(part 1 of 2)
# Autodesk Inventor assembly: NewChassis
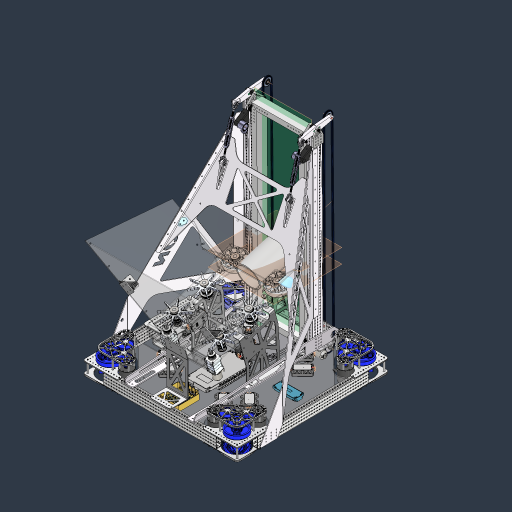
[picture p0: Inventor's stored thumbnail of the model, 512x512]
Saved by Autodesk Inventor 2024.3 (Build 283343000, 343)
## iProperties
ILogicPurgeVersion: 0.0.0.0
OnSaveVersion: 3.4.3.0
OnSaveAssembly: COREAutomationManager
Created: 2025-01-13
Part Number: NewChassis
Document SubType Name: Assembly
Designer: Marcus Tannini
Mfg Approved By: John.Thibert
Mass: 38555.3 g
Surface Area: 112070 cm^2
Volume: 16960.9 cm^3
Density: 2.27319 g/cm^3
ModelCat: Uncategorized
CN_MASS: 40.55
Author: Marcus Tannini
## Documents named in this file (68)
- C:\Users\Marcus Tannini\Documents\GitHub\2025-Poseidon-Mechanical\#Poseidon 2025.iam
- C:\Users\Marcus Tannini\Documents\GitHub\2025-Poseidon-Mechanical\ASSY,MK4i,Swerve_Module_INV.iam
- C:\Users\Marcus Tannini\Documents\GitHub\2025-Poseidon-Mechanical\MAXTube-2x1-Holes.ipt
- C:\Users\Marcus Tannini\Documents\GitHub\2025-Poseidon-Mechanical\BellyPanTop.ipt
- C:\Users\Marcus Tannini\Documents\GitHub\2025-Poseidon-Mechanical\BellyPanBot.ipt
- C:\Users\Marcus Tannini\Documents\GitHub\2025-Poseidon-Mechanical\BATTERY,12V.ipt
- C:\Users\Marcus Tannini\Documents\GitHub\2025-Poseidon-Mechanical\CONTROLS,MAIN_BREAKER.ipt
- C:\Users\Marcus Tannini\Documents\GitHub\2025-Poseidon-Mechanical\CONTROLS,MOTOR,NEO,550.ipt
- C:\Users\Marcus Tannini\Documents\GitHub\2025-Poseidon-Mechanical\CONTROLS,PDH.ipt
- C:\Users\Marcus Tannini\Documents\GitHub\2025-Poseidon-Mechanical\CONTROLS,PH.ipt
- C:\Users\Marcus Tannini\Documents\GitHub\2025-Poseidon-Mechanical\CONTROLS,ROBO_RIO.ipt
- C:\Users\Marcus Tannini\Documents\GitHub\2025-Poseidon-Mechanical\CONTROLS,SPARK_MAX.ipt
- C:\Users\Marcus Tannini\Documents\GitHub\2025-Poseidon-Mechanical\CONTROLS,VRM.ipt
- C:\Users\Marcus Tannini\Documents\GitHub\2025-Poseidon-Mechanical\COVER,SPARKMAX.ipt
- C:\Users\Marcus Tannini\Documents\GitHub\2025-Poseidon-Mechanical\ModifiedCase(IncludesPatterning).iam
- C:\Users\Marcus Tannini\Documents\GitHub\2025-Poseidon-Mechanical\PLATE,MOUNT,BATTERY,TOP.ipt
- C:\Users\Marcus Tannini\Documents\GitHub\2025-Poseidon-Mechanical\PLATE,MOUNT,BATTERY,BOT.ipt
- C:\Users\Marcus Tannini\Documents\GitHub\2025-Poseidon-Mechanical\MOUNT,STRAP,BATTERY.ipt
- C:\Users\Marcus Tannini\Documents\GitHub\2025-Poseidon-Mechanical\SPACER,SPROCKET,IDLER,ELEVATOR.ipt
- C:\Users\Marcus Tannini\Documents\GitHub\2025-Poseidon-Mechanical\22.ipt
- C:\Users\Marcus Tannini\Documents\GitHub\2025-Poseidon-Mechanical\PLATE,MOUNT,DRIVE,ELEVATOR.ipt
- C:\Users\Marcus Tannini\Documents\GitHub\2025-Poseidon-Mechanical\PLATE,BEARING,DRIVE,ELEVATOR.ipt
- C:\Users\Marcus Tannini\Documents\GitHub\2025-Poseidon-Mechanical\PURCHASED,HEX_BEARING.ipt
- C:\Users\Marcus Tannini\Documents\GitHub\2025-Poseidon-Mechanical\SHAFT,HEX,0.500in,DRIVE,ELEVATOR.ipt
- C:\Users\Marcus Tannini\Documents\GitHub\2025-Poseidon-Mechanical\PLATE,SIDE,BRACE,RIGHT,ELEVATOR.ipt
- C:\Users\Marcus Tannini\Documents\GitHub\2025-Poseidon-Mechanical\PLATE,SIDE,BRACE,LEFT,ELEVATOR.ipt
- C:\Users\Marcus Tannini\Documents\GitHub\2025-Poseidon-Mechanical\PLATE,TURNBUCKLE,TENSIONER,CHAIN.ipt
- C:\Users\Marcus Tannini\Documents\GitHub\2025-Poseidon-Mechanical\PLATE,BRACE,HORISONTAL,TOP,ELEVATOR.ipt
- C:\Users\Marcus Tannini\Documents\GitHub\2025-Poseidon-Mechanical\TURNBUCKLE,0.25IN_CLEVIS.iam
- C:\Users\Marcus Tannini\Documents\GitHub\2025-Poseidon-Mechanical\STAGE1,ELEVATOR.iam
- C:\Users\Marcus Tannini\Documents\GitHub\2025-Poseidon-Mechanical\ASSY,MAIN,ELEVATOR.iam
- C:\Users\Marcus Tannini\Documents\GitHub\2025-Poseidon-Mechanical\ANGLE,MOUNT,ELEVATOR.ipt
- C:\Users\Marcus Tannini\Documents\GitHub\2025-Poseidon-Mechanical\ANGLE,MOUNT,ELEVATOR,MIRR.ipt
- C:\Users\Marcus Tannini\Documents\GitHub\2025-Poseidon-Mechanical\FABRIC,BUMPERS.ipt
- C:\Users\Marcus Tannini\Documents\GitHub\2025-Poseidon-Mechanical\9293K119_Constant-Force Spring.ipt
- C:\Users\Marcus Tannini\Documents\GitHub\2025-Poseidon-Mechanical\MOUNT,SPRING,ELEVATOR.ipt
- C:\Users\Marcus Tannini\Documents\GitHub\2025-Poseidon-Mechanical\MOUNT,SPRING,ELEVATOR,MIRR.ipt
- C:\Users\Marcus Tannini\Documents\GitHub\2025-Poseidon-Mechanical\VersaPlanetary v2 Dual Stage 10_1 with RS 550 (1).iam
- C:\Users\Marcus Tannini\Documents\GitHub\2025-Poseidon-Mechanical\hopper_side_l.ipt
- C:\Users\Marcus Tannini\Documents\GitHub\2025-Poseidon-Mechanical\hopper_side_r.ipt
- C:\Users\Marcus Tannini\Documents\GitHub\2025-Poseidon-Mechanical\hopper_back.ipt
- C:\Users\Marcus Tannini\Documents\GitHub\2025-Poseidon-Mechanical\feeder_bottom_plate.ipt
- C:\Users\Marcus Tannini\Documents\GitHub\2025-Poseidon-Mechanical\hopper_side_bracket.ipt
- C:\Users\Marcus Tannini\Documents\GitHub\2025-Poseidon-Mechanical\feeder_guide_plate.ipt
- C:\Users\Marcus Tannini\Documents\GitHub\2025-Poseidon-Mechanical\am-5123 5IN 500IN Hex Bore Compliant Star.iam
- C:\Users\Marcus Tannini\Documents\GitHub\2025-Poseidon-Mechanical\feeder_guide_plate_MIR.ipt
- C:\Users\Marcus Tannini\Documents\GitHub\2025-Poseidon-Mechanical\feeder_front_support.ipt
- C:\Users\Marcus Tannini\Documents\GitHub\2025-Poseidon-Mechanical\Coral.ipt
- C:\Users\Marcus Tannini\Documents\GitHub\2025-Poseidon-Mechanical\coral_guide.ipt
- C:\Users\Marcus Tannini\Documents\GitHub\2025-Poseidon-Mechanical\coral_guide_MIR.ipt
- C:\Users\Marcus Tannini\Documents\GitHub\2025-Poseidon-Mechanical\hopper_back_support.ipt
- C:\Users\Marcus Tannini\Documents\GitHub\2025-Poseidon-Mechanical\feeder_side_support_r.ipt
- C:\Users\Marcus Tannini\Documents\GitHub\2025-Poseidon-Mechanical\feeder_side_support_l.ipt
- C:\Users\Marcus Tannini\Documents\GitHub\2025-Poseidon-Mechanical\feeder_middle_brace.ipt
- C:\Users\Marcus Tannini\Documents\GitHub\2025-Poseidon-Mechanical\2_1-2_hex_shaft.ipt
- C:\Users\Marcus Tannini\Documents\GitHub\2025-Poseidon-Mechanical\Bolt_Spacer.ipt
- C:\Users\Marcus Tannini\Documents\GitHub\2025-Poseidon-Mechanical\hopper_backboard.ipt
- C:\Users\Marcus Tannini\Documents\GitHub\2025-Poseidon-Mechanical\16t 9mm.ipt
- C:\Users\Marcus Tannini\Documents\GitHub\2025-Poseidon-Mechanical\19t 9mm.ipt
- C:\Users\Marcus Tannini\Documents\GitHub\2025-Poseidon-Mechanical\29t 9mm.ipt
- C:\Users\Marcus Tannini\Documents\GitHub\2025-Poseidon-Mechanical\coral_end_stop.ipt
- C:\Users\Marcus Tannini\Documents\GitHub\2025-Poseidon-Mechanical\coral_end_stop_MIR.ipt
- C:\Users\Marcus Tannini\Documents\GitHub\2025-Poseidon-Mechanical\Part Studio 1 - Support 1.ipt
- C:\Users\Marcus Tannini\Documents\GitHub\2025-Poseidon-Mechanical\Part Studio 1 - Support 2.ipt
- C:\Users\Marcus Tannini\Documents\GitHub\2025-Poseidon-Mechanical\am-3480 4IN 500Hex Bore Compliant Wheel REV2(1).iam
- C:\Users\Marcus Tannini\Documents\GitHub\2025-Poseidon-Mechanical\1-2in_spacer.ipt
- C:\Users\Marcus Tannini\Documents\GitHub\2025-Poseidon-Mechanical\hopper_fin.ipt
- C:\Users\Marcus Tannini\Documents\GitHub\2025-Poseidon-Mechanical\hopper_fin_MIR.ipt
## Components (143 placed, 70 different names)
1. FABRIC,BUMPERS.ipt:1 — Flush:323, Mate:335, Mate:336
2. am-3480 4IN 500Hex Bore Compliant Wheel REV2(1):1 [sub-assembly] — Mate:717, Mate:718, Mate:719, Mate:725
3. am-3480 4IN 500Hex Bore Compliant Wheel REV2(1):2 [sub-assembly] — Mate:720, Mate:721, Mate:722
4. 1-2in_spacer:1 — Mate:723, Mate:724, Mate:725
5. 1-2in_spacer:2 — Mate:726, Mate:727, Mate:728
6. 1-2in_spacer:3 — Mate:729, Mate:730, Mate:731
7. 1-2in_spacer:4 — Mate:738, Mate:739, Mate:740
8. 1-2in_spacer:5 — Mate:735, Mate:736, Mate:737
9. 1-2in_spacer:6 — Mate:732, Mate:733, Mate:734
10. hopper_fin:1 — Mate:749, Mate:750, Mate:754
11. hopper_fin_MIR:1 — Mate:751, Mate:752, Mate:753
12. BellyPanBot.ipt:1 — Mate:66, Mate:353, Mate:354
13. BellyPanTop.ipt:1 — Mate:62, Mate:63, Mate:65, Mate:70, Mate:71, Mate:82, Mate:84, Insert:7, Insert:8, Insert:9, Insert:10, Insert:11, Insert:12, Insert:13, Insert:14, Insert:15, Insert:16, Insert:17, Insert:18, Insert:19, Insert:20, Insert:21, Insert:22, Mate:111, Mate:113, Mate:114, Mate:116, Mate:117, Mate:118, Mate:119, Mate:121, Mate:122, Mate:123, Mate:124, Mate:125, Mate:126, Mate:127, Mate:130, Insert:23, Insert:24, Mate:223, Mate:308, Mate:320, Mate:349, Mate:350, Angle:11, Mate:541, Mate:542, Mate:544, Mate:548, Flush:336, Mate:549
14. MAXTube-2x1-Holes.ipt:1 — Mate:1, Mate:2, Mate:3, Mate:4, Mate:5, Mate:15, Mate:115, Mate:272
15. MAXTube-2x1-Holes.ipt:2 — Mate:6, Mate:7, Mate:8, Mate:9, Mate:10, Mate:11, Mate:62, Flush:17, Mate:309, Mate:310, Mate:542, Mate:543
16. MAXTube-2x1-Holes.ipt:3 — Mate:19, Mate:20, Mate:21, Mate:66, Mate:114, Mate:312, Mate:313, Mate:336
17. MAXTube-2x1-Holes.ipt:4 — Mate:12, Mate:13, Mate:14, Mate:16, Mate:17, Mate:18, Mate:29, Mate:63, Mate:271, Mate:353, Mate:354
18. MOUNT,STRAP,BATTERY.ipt:1 — Mate:357, Mate:358, Mate:359
19. PLATE,MOUNT,BATTERY,BOT.ipt:1 — Mate:320, Mate:321, Mate:351, Mate:352
20. PLATE,MOUNT,BATTERY,TOP.ipt:1 — Mate:127, Mate:349, Mate:350, Mate:351, Mate:352, Mate:356, Mate:357, Mate:358, Mate:359
21. BATTERY,12V.ipt:1 — Mate:321, Mate:356
22. CONTROLS,MAIN_BREAKER.ipt:1 — Mate:82, Mate:111, Mate:116
23. CONTROLS,PDH.ipt:1 — Mate:113, Mate:117, Mate:118, Mate:119
24. CONTROLS,PH.ipt:1 — Insert:23, Insert:24
25. CONTROLS,ROBO_RIO.ipt:1 — Mate:124, Mate:125, Mate:126
26. CONTROLS,SPARK_MAX.ipt:1 — Mate:84, Mate:85, Mate:86, Mate:87
27. CONTROLS,VRM.ipt:1 — Mate:121, Mate:122, Mate:123
28. ModifiedCase(IncludesPatterning).iam:1 [sub-assembly] — Mate:130
29. ASSY,MK4i,Swerve_Module_INV.iam:1 [sub-assembly] — Mate:1, Mate:2, Mate:15
30. ASSY,MK4i,Swerve_Module_INV.iam:2 [sub-assembly] — Mate:3, Mate:4, Mate:5, Mate:6, Mate:7, Mate:8
31. ASSY,MK4i,Swerve_Module_INV.iam:3 [sub-assembly] — Mate:9, Mate:10, Mate:11, Mate:12, Mate:13, Mate:14
32. ASSY,MK4i,Swerve_Module_INV.iam:4 [sub-assembly] — Mate:16, Mate:17, Mate:18, Mate:19, Mate:20, Mate:21, Mate:67
33. CONTROLS,SPARK_MAX.ipt:2
34. CONTROLS,SPARK_MAX.ipt:3
35. CONTROLS,SPARK_MAX.ipt:4
36. CONTROLS,SPARK_MAX.ipt:5
37. CONTROLS,SPARK_MAX.ipt:6
38. CONTROLS,SPARK_MAX.ipt:7
39. CONTROLS,SPARK_MAX.ipt:8
40. COVER,SPARKMAX.ipt:1 — Mate:85, Mate:86, Mate:87, Insert:7, Insert:8
41. COVER,SPARKMAX.ipt:2 — Insert:9, Insert:10
42. COVER,SPARKMAX.ipt:3 — Insert:11, Insert:12
43. COVER,SPARKMAX.ipt:4 — Insert:13, Insert:14
44. COVER,SPARKMAX.ipt:5 — Insert:17, Insert:18
45. COVER,SPARKMAX.ipt:6 — Insert:15, Insert:16
46. COVER,SPARKMAX.ipt:7 — Insert:21, Insert:22
47. COVER,SPARKMAX.ipt:8 — Insert:19, Insert:20
48. 9293K119_Constant-Force Spring:1 — Mate:364, Mate:365
49. 9293K119_Constant-Force Spring:2 — Mate:370, Mate:371
50. MOUNT,SPRING,ELEVATOR:1 — Mate:363, Mate:362, Mate:364, Mate:365, Mate:366
51. MOUNT,SPRING,ELEVATOR,MIRR:1 — Mate:367, Mate:368, Mate:369, Mate:370, Mate:371
52. CONTROLS,MOTOR,NEO,550:3
53. VersaPlanetary v2 Dual Stage 10_1 with RS 550 (1):1 [sub-assembly] — Mate:472, Mate:473, Mate:474
54. CONTROLS,MOTOR,NEO,550:4
55. VersaPlanetary v2 Dual Stage 10_1 with RS 550 (1):2 [sub-assembly] — Mate:469, Mate:470, Mate:471
56. ASSY,MAIN,ELEVATOR.iam:1 [sub-assembly] — Mate:161, Mate:162, Flush:19, Mate:297, STAGE1 UPPER LIMIT, STAGE1 MAX, Mate:311, Mate:314, Mate:315, Mate:363, Mate:362, Mate:366, Mate:367, Mate:368, Mate:369
57. STAGE1,ELEVATOR.iam:1 [sub-assembly] — Flush:19, Mate:297, STAGE1 LOWER LIMIT, STAGE1 UPPER LIMIT, STAGE1 MIN, STAGE1 MAX
58. 22.ipt:1 — Mate:227, Angle:6
59. 22.ipt:2 — Mate:233, Angle:4, Flush:14
60. ANGLE,MOUNT,ELEVATOR.ipt:1 — Mate:65, Mate:70, Mate:71, Mate:161, Mate:162, Mate:224, STAGE1 LOWER LIMIT, STAGE1 MIN, Flush:337, Mate:556
61. ANGLE,MOUNT,ELEVATOR,MIRR.ipt:1 — Mate:308, Mate:309, Mate:310, Mate:311, Mate:312, Mate:313, Mate:314, Mate:315, Flush:329, Angle:12, Mate:550, Mate:551, Mate:552
62. PLATE,BEARING,DRIVE,ELEVATOR.ipt:1 — Mate:226, Mate:227, Mate:228, Mate:229, Insert:50
63. PLATE,BEARING,DRIVE,ELEVATOR.ipt:2 — Mate:230, Mate:231, Mate:232, Insert:49, Mate:233, Mate:234
64. PLATE,BRACE,HORISONTAL,TOP,ELEVATOR.ipt:1 — Mate:285, Mate:286, Mate:289, Mate:290, Mate:291, Mate:295, Mate:296, Mate:714, Mate:746, Mate:747, Mate:748
65. PLATE,MOUNT,DRIVE,ELEVATOR.ipt:1 — Mate:223, Mate:224, Mate:226, Mate:228, Mate:229, Mate:230, Mate:231, Mate:232, Flush:329, Mate:469, Mate:470, Mate:471, Mate:472, Mate:473, Mate:474
66. PLATE,SIDE,BRACE,LEFT,ELEVATOR.ipt:1 — Mate:271, Mate:289, Mate:290, Mate:291, Mate:335
67. PLATE,SIDE,BRACE,RIGHT,ELEVATOR.ipt:1 — Mate:272
68. PLATE,TURNBUCKLE,TENSIONER,CHAIN.ipt:1 — Mate:285, Mate:296
69. PLATE,TURNBUCKLE,TENSIONER,CHAIN.ipt:2 — Mate:286, Mate:295
70. PURCHASED,HEX_BEARING.ipt:1 — Insert:49, Angle:5
71. PURCHASED,HEX_BEARING.ipt:2 — Insert:50, Angle:7
72. SHAFT,HEX,0.500in,DRIVE,ELEVATOR.ipt:1 — Mate:234, Angle:4, Angle:5, Angle:6, Angle:7, Flush:14
73. SPACER,SPROCKET,IDLER,ELEVATOR.ipt:1
74. SPACER,SPROCKET,IDLER,ELEVATOR.ipt:2
75. TURNBUCKLE,0.25IN_CLEVIS.iam:1 [sub-assembly]
76. TURNBUCKLE,0.25IN_CLEVIS.iam:2 [sub-assembly]
77. Part Studio 1 - Support 2:1 — Mate:743, Mate:744, Mate:745
78. Part Studio 1 - Support 1:1 — Mate:713, Mate:714
79. coral_end_stop_MIR:1 — Flush:364, Mate:715, Flush:365
80. coral_end_stop:1 — Mate:704, Flush:362, Flush:364, Mate:715, Flush:365, Mate:716
81. hopper_side_l:1 — Mate:496, Mate:497, Mate:498, Mate:743, Mate:744, Mate:745
82. hopper_side_r:1 — Mate:502, Mate:503, Mate:504, Mate:713
83. feeder_bottom_plate:1 — Angle:11, Mate:490, Mate:491, Mate:492, Mate:507, Mate:512, Mate:519, Mate:534, Angle:12, Flush:333, Mate:537, Flush:334, Mate:539, Flush:335, Mate:545, Mate:546, Mate:547, Mate:577, Mate:578, Mate:605, Mate:608, Mate:609, Mate:610, Mate:611, Mate:630, Mate:631, Mate:632, Mate:633, Mate:634, Mate:646, Mate:647, Mate:648, Mate:649, Mate:656, Mate:657, Mate:658, Mate:659, Mate:698, Mate:700, Mate:741, Mate:742
84. hopper_back:1 — Mate:490, Mate:491, Mate:492, Mate:493, Mate:494, Mate:495, Mate:499, Mate:500, Mate:501, Mate:749, Mate:750, Mate:751, Mate:752, Mate:753, Mate:754
85. hopper_side_bracket:1 — Mate:493, Mate:494, Mate:495, Mate:496, Mate:497, Mate:498
86. hopper_side_bracket:2 — Mate:499, Mate:500, Mate:501, Mate:502, Mate:503, Mate:504
87. feeder_guide_plate:1 — Mate:507, Mate:577, Mate:644, Mate:645, Mate:650, Mate:651, Mate:652, Mate:653, Mate:699, Mate:742
88. am-5123 5IN 500IN Hex Bore Compliant Star:2 [sub-assembly] — Flush:353, Mate:654, Mate:655, Flush:354, Mate:731
89. feeder_guide_plate_MIR:1 — Mate:512, Mate:520, Mate:578, Mate:660, Mate:661, Mate:662, Mate:663, Mate:664, Mate:665, Mate:701, Mate:741
90. feeder_front_support:1 — Mate:541, Mate:543, Mate:544, Mate:704, Flush:362, Mate:716
91. Coral:1 — Mate:519, Mate:520, Mate:630
92. CONTROLS,MOTOR,NEO,550:5
93. VersaPlanetary v2 Dual Stage 10_1 with RS 550 (1):3 [sub-assembly] — Mate:534, Mate:631, Mate:632, Mate:668, Mate:670
94. coral_guide:1 — Flush:333, Mate:537, Mate:540, Flush:335
95. coral_guide_MIR:1 — Flush:334, Mate:539, Mate:540
96. hopper_back_support:1 — Mate:545, Mate:546, Mate:547, Mate:548, Flush:336, Mate:549
97. feeder_side_support_r:1 — Flush:337, Mate:553, Mate:554, Mate:555, Mate:556, Mate:624, Mate:625, Mate:626
98. feeder_side_support_l:1 — Mate:550, Mate:551, Mate:552, Mate:627, Mate:628, Mate:629
99. feeder_middle_brace:1 — Mate:553, Mate:554, Mate:555
100. 2_1-2_hex_shaft:1 — Mate:557, Mate:558, Flush:340, Mate:561, Mate:562, Rotation:4, Rotation:5, Mate:685, Mate:686, Mate:688, Mate:689, Mate:726, Mate:727
101. PURCHASED,HEX_BEARING:3 — Mate:557, Mate:558, Flush:340, Mate:573, Mate:652, Mate:653
102. 2_1-2_hex_shaft:2 — Rotation:5, Mate:690, Mate:691, Mate:717, Mate:718, Mate:723, Mate:724
103. PURCHASED,HEX_BEARING:4 — Mate:650, Mate:651, Mate:719
104. am-5123 5IN 500IN Hex Bore Compliant Star:3 [sub-assembly] — Mate:561, Mate:562, Mate:573, Flush:353
105. 2_1-2_hex_shaft:3 — Rotation:1, Rotation:2, Mate:680, Mate:681, Mate:693, Mate:694, Mate:735, Mate:736
106. PURCHASED,HEX_BEARING:5 — Mate:660, Mate:661
107. am-5123 5IN 500IN Hex Bore Compliant Star:5 [sub-assembly]
108. 2_1-2_hex_shaft:4 — Rotation:2, Mate:695, Mate:696, Mate:720, Mate:721, Mate:738, Mate:739
109. PURCHASED,HEX_BEARING:6 — Mate:662, Mate:663, Mate:722
110. am-5123 5IN 500IN Hex Bore Compliant Star:7 [sub-assembly] — Mate:666, Mate:667, Flush:354
111. CONTROLS,MOTOR,NEO,550:6
112. VersaPlanetary v2 Dual Stage 10_1 with RS 550 (1):4 [sub-assembly] — Mate:605, Mate:633, Mate:634, Mate:673, Mate:674
113. PURCHASED,HEX_BEARING:7 — Mate:648, Mate:649
114. PURCHASED,HEX_BEARING:8 — Mate:646, Mate:647
115. PURCHASED,HEX_BEARING:9 — Mate:658, Mate:659
116. PURCHASED,HEX_BEARING:10 — Mate:656, Mate:657
117. Bolt_Spacer:1 — Mate:608, Mate:609
118. Bolt_Spacer:2 — Mate:610, Mate:611
119. hopper_backboard:1 — Mate:746, Mate:747, Mate:748
120. CONTROLS,SPARK_MAX:9 — Mate:626
121. COVER,SPARKMAX:9 — Mate:624, Mate:625
122. CONTROLS,SPARK_MAX:10 — Mate:629
123. COVER,SPARKMAX:10 — Mate:627, Mate:628
124. PURCHASED,HEX_BEARING:11 — Mate:636, Mate:637, Flush:349, Mate:664, Mate:665
125. 2_1-2_hex_shaft:5 — Flush:351, Mate:640, Mate:641, Flush:352, Mate:642, Mate:643, Mate:654, Mate:655, Rotation:3, Rotation:4, Mate:671, Mate:672, Mate:682, Mate:684, Mate:729, Mate:730
126. 2_1-2_hex_shaft:6 — Mate:636, Mate:637, Flush:349, Flush:350, Mate:638, Mate:639, Mate:666, Mate:667, Rotation:1, Rotation:3, Mate:675, Mate:676, Mate:678, Mate:679, Mate:732, Mate:733
127. PURCHASED,HEX_BEARING:12 — Flush:351, Mate:640, Mate:641, Mate:644, Mate:645
128. PURCHASED,HEX_BEARING:13 — Flush:352, Mate:642, Mate:643
129. PURCHASED,HEX_BEARING:14 — Flush:350, Mate:638, Mate:639, Mate:697
130. 16t 9mm:1 — Mate:671, Mate:672, Flush:355, Mate:683
131. 16t 9mm:2 — Mate:668, Mate:670, Flush:355, Flush:356
132. 16t 9mm:3 — Mate:673, Mate:674, Flush:356, Flush:357
133. 16t 9mm:4 — Mate:675, Mate:676, Flush:357, Mate:677, Mate:697
134. 19t 9mm:1 — Mate:682, Mate:683, Mate:684, Flush:359
135. 19t 9mm:2 — Mate:680, Flush:358, Mate:681, Mate:692, Mate:737
136. 19t 9mm:3 — Mate:678, Mate:677, Mate:679, Flush:358, Mate:734
137. 19t 9mm:4 — Mate:685, Flush:359, Mate:686, Mate:687, Mate:728
138. 29t 9mm:1 — Flush:360, Mate:690, Mate:691
139. 29t 9mm:2 — Mate:687, Mate:688, Mate:689, Flush:360
140. 29t 9mm:3 — Mate:692, Mate:693, Mate:694, Flush:361
141. 29t 9mm:4 — Flush:361, Mate:695, Mate:696, Mate:740
142. Bolt_Spacer:3 — Mate:698, Mate:699
143. Bolt_Spacer:4 — Mate:700, Mate:701
## Relationships (411: Mate 342, Flush 34, Insert 24, Angle 6, RelateRotation 5)
- Mate:1: MAXTube-2x1-Holes.ipt:1 ↔ ASSY,MK4i,Swerve_Module_INV.iam:1
- Mate:2: MAXTube-2x1-Holes.ipt:1 ↔ ASSY,MK4i,Swerve_Module_INV.iam:1
- Mate:3: MAXTube-2x1-Holes.ipt:1 ↔ ASSY,MK4i,Swerve_Module_INV.iam:2
- Mate:4: MAXTube-2x1-Holes.ipt:1 ↔ ASSY,MK4i,Swerve_Module_INV.iam:2
- Mate:5: MAXTube-2x1-Holes.ipt:1 ↔ ASSY,MK4i,Swerve_Module_INV.iam:2
- Mate:6: MAXTube-2x1-Holes.ipt:2 ↔ ASSY,MK4i,Swerve_Module_INV.iam:2
- Mate:7: MAXTube-2x1-Holes.ipt:2 ↔ ASSY,MK4i,Swerve_Module_INV.iam:2
- Mate:8: MAXTube-2x1-Holes.ipt:2 ↔ ASSY,MK4i,Swerve_Module_INV.iam:2
- Mate:9: MAXTube-2x1-Holes.ipt:2 ↔ ASSY,MK4i,Swerve_Module_INV.iam:3
- Mate:10: MAXTube-2x1-Holes.ipt:2 ↔ ASSY,MK4i,Swerve_Module_INV.iam:3
- Mate:11: MAXTube-2x1-Holes.ipt:2 ↔ ASSY,MK4i,Swerve_Module_INV.iam:3
- Mate:12: MAXTube-2x1-Holes.ipt:4 ↔ ASSY,MK4i,Swerve_Module_INV.iam:3
- Mate:13: MAXTube-2x1-Holes.ipt:4 ↔ ASSY,MK4i,Swerve_Module_INV.iam:3
- Mate:14: MAXTube-2x1-Holes.ipt:4 ↔ ASSY,MK4i,Swerve_Module_INV.iam:3
- Mate:15: MAXTube-2x1-Holes.ipt:1 ↔ ASSY,MK4i,Swerve_Module_INV.iam:1
- Mate:16: MAXTube-2x1-Holes.ipt:4 ↔ ASSY,MK4i,Swerve_Module_INV.iam:4
- Mate:17: MAXTube-2x1-Holes.ipt:4 ↔ ASSY,MK4i,Swerve_Module_INV.iam:4
- Mate:18: MAXTube-2x1-Holes.ipt:4 ↔ ASSY,MK4i,Swerve_Module_INV.iam:4
- Mate:19: MAXTube-2x1-Holes.ipt:3 ↔ ASSY,MK4i,Swerve_Module_INV.iam:4
- Mate:20: MAXTube-2x1-Holes.ipt:3 ↔ ASSY,MK4i,Swerve_Module_INV.iam:4
- Mate:21: MAXTube-2x1-Holes.ipt:3 ↔ ASSY,MK4i,Swerve_Module_INV.iam:4
- Mate:29 (-6.35 mm): MAXTube-2x1-Holes.ipt:4
- Mate:62: BellyPanTop.ipt:1 ↔ MAXTube-2x1-Holes.ipt:2
- Mate:63: BellyPanTop.ipt:1 ↔ MAXTube-2x1-Holes.ipt:4
- Mate:65: BellyPanTop.ipt:1 ↔ ANGLE,MOUNT,ELEVATOR.ipt:1
- Mate:66: BellyPanBot.ipt:1 ↔ MAXTube-2x1-Holes.ipt:3
- Mate:67 (35.56 mm): ASSY,MK4i,Swerve_Module_INV.iam:4
- Mate:70: BellyPanTop.ipt:1 ↔ ANGLE,MOUNT,ELEVATOR.ipt:1
- Mate:71: BellyPanTop.ipt:1 ↔ ANGLE,MOUNT,ELEVATOR.ipt:1
- Mate:321: PLATE,MOUNT,BATTERY,BOT.ipt:1 ↔ BATTERY,12V.ipt:1
- Mate:82: BellyPanTop.ipt:1 ↔ CONTROLS,MAIN_BREAKER.ipt:1
- Mate:84: BellyPanTop.ipt:1 ↔ CONTROLS,SPARK_MAX.ipt:1
- Mate:85: CONTROLS,SPARK_MAX.ipt:1 ↔ COVER,SPARKMAX.ipt:1
- Mate:86: CONTROLS,SPARK_MAX.ipt:1 ↔ COVER,SPARKMAX.ipt:1
- Mate:87: CONTROLS,SPARK_MAX.ipt:1 ↔ COVER,SPARKMAX.ipt:1
- Insert:7: BellyPanTop.ipt:1 ↔ COVER,SPARKMAX.ipt:1
- Insert:8: BellyPanTop.ipt:1 ↔ COVER,SPARKMAX.ipt:1
- [Mate]: CONTROLS,SPARK_MAX.ipt:2 ↔ COVER,SPARKMAX.ipt:2
- [Mate]: CONTROLS,SPARK_MAX.ipt:2 ↔ COVER,SPARKMAX.ipt:2
- [Mate]: CONTROLS,SPARK_MAX.ipt:2 ↔ COVER,SPARKMAX.ipt:2
- [Mate]: CONTROLS,SPARK_MAX.ipt:3 ↔ COVER,SPARKMAX.ipt:3
- [Mate]: CONTROLS,SPARK_MAX.ipt:3 ↔ COVER,SPARKMAX.ipt:3
- [Mate]: CONTROLS,SPARK_MAX.ipt:3 ↔ COVER,SPARKMAX.ipt:3
- [Mate]: CONTROLS,SPARK_MAX.ipt:4 ↔ COVER,SPARKMAX.ipt:4
- [Mate]: CONTROLS,SPARK_MAX.ipt:4 ↔ COVER,SPARKMAX.ipt:4
- [Mate]: CONTROLS,SPARK_MAX.ipt:4 ↔ COVER,SPARKMAX.ipt:4
- [Mate]: CONTROLS,SPARK_MAX.ipt:5 ↔ COVER,SPARKMAX.ipt:5
- [Mate]: CONTROLS,SPARK_MAX.ipt:5 ↔ COVER,SPARKMAX.ipt:5
- [Mate]: CONTROLS,SPARK_MAX.ipt:5 ↔ COVER,SPARKMAX.ipt:5
- [Mate]: CONTROLS,SPARK_MAX.ipt:6 ↔ COVER,SPARKMAX.ipt:6
- [Mate]: CONTROLS,SPARK_MAX.ipt:6 ↔ COVER,SPARKMAX.ipt:6
- [Mate]: CONTROLS,SPARK_MAX.ipt:6 ↔ COVER,SPARKMAX.ipt:6
- [Mate]: CONTROLS,SPARK_MAX.ipt:7 ↔ COVER,SPARKMAX.ipt:7
- [Mate]: CONTROLS,SPARK_MAX.ipt:7 ↔ COVER,SPARKMAX.ipt:7
- [Mate]: CONTROLS,SPARK_MAX.ipt:7 ↔ COVER,SPARKMAX.ipt:7
- [Mate]: CONTROLS,SPARK_MAX.ipt:8 ↔ COVER,SPARKMAX.ipt:8
- [Mate]: CONTROLS,SPARK_MAX.ipt:8 ↔ COVER,SPARKMAX.ipt:8
- [Mate]: CONTROLS,SPARK_MAX.ipt:8 ↔ COVER,SPARKMAX.ipt:8
- Insert:9: BellyPanTop.ipt:1 ↔ COVER,SPARKMAX.ipt:2
- Insert:10: BellyPanTop.ipt:1 ↔ COVER,SPARKMAX.ipt:2
- Insert:11: BellyPanTop.ipt:1 ↔ COVER,SPARKMAX.ipt:3
- Insert:12: BellyPanTop.ipt:1 ↔ COVER,SPARKMAX.ipt:3
- Insert:13: BellyPanTop.ipt:1 ↔ COVER,SPARKMAX.ipt:4
- Insert:14: BellyPanTop.ipt:1 ↔ COVER,SPARKMAX.ipt:4
- Insert:15: BellyPanTop.ipt:1 ↔ COVER,SPARKMAX.ipt:6
- Insert:16: BellyPanTop.ipt:1 ↔ COVER,SPARKMAX.ipt:6
- Insert:17: BellyPanTop.ipt:1 ↔ COVER,SPARKMAX.ipt:5
- Insert:18: BellyPanTop.ipt:1 ↔ COVER,SPARKMAX.ipt:5
- Insert:19: BellyPanTop.ipt:1 ↔ COVER,SPARKMAX.ipt:8
- Insert:20: BellyPanTop.ipt:1 ↔ COVER,SPARKMAX.ipt:8
- Insert:21: BellyPanTop.ipt:1 ↔ COVER,SPARKMAX.ipt:7
- Insert:22: BellyPanTop.ipt:1 ↔ COVER,SPARKMAX.ipt:7
- Mate:111: BellyPanTop.ipt:1 ↔ CONTROLS,MAIN_BREAKER.ipt:1
- Mate:113: BellyPanTop.ipt:1 ↔ CONTROLS,PDH.ipt:1
- Mate:114: BellyPanTop.ipt:1 ↔ MAXTube-2x1-Holes.ipt:3
- Mate:115 (-374.65 mm): MAXTube-2x1-Holes.ipt:1
- Mate:116 (0.254 mm): BellyPanTop.ipt:1 ↔ CONTROLS,MAIN_BREAKER.ipt:1
- Mate:117: BellyPanTop.ipt:1 ↔ CONTROLS,PDH.ipt:1
- Mate:118: BellyPanTop.ipt:1 ↔ CONTROLS,PDH.ipt:1
- Mate:119: BellyPanTop.ipt:1 ↔ CONTROLS,PDH.ipt:1
- Mate:121: BellyPanTop.ipt:1 ↔ CONTROLS,VRM.ipt:1
- Mate:122: BellyPanTop.ipt:1 ↔ CONTROLS,VRM.ipt:1
- Mate:123: BellyPanTop.ipt:1 ↔ CONTROLS,VRM.ipt:1
- Mate:124: BellyPanTop.ipt:1 ↔ CONTROLS,ROBO_RIO.ipt:1
- Mate:125: BellyPanTop.ipt:1 ↔ CONTROLS,ROBO_RIO.ipt:1
- Mate:126: BellyPanTop.ipt:1 ↔ CONTROLS,ROBO_RIO.ipt:1
- Mate:127: BellyPanTop.ipt:1 ↔ PLATE,MOUNT,BATTERY,TOP.ipt:1
- Mate:130: BellyPanTop.ipt:1 ↔ ModifiedCase(IncludesPatterning).iam:1
- Insert:23: BellyPanTop.ipt:1 ↔ CONTROLS,PH.ipt:1
- Insert:24: BellyPanTop.ipt:1 ↔ CONTROLS,PH.ipt:1
- Mate:161: ASSY,MAIN,ELEVATOR.iam:1 ↔ ANGLE,MOUNT,ELEVATOR.ipt:1
- Mate:162: ASSY,MAIN,ELEVATOR.iam:1 ↔ ANGLE,MOUNT,ELEVATOR.ipt:1
- [Mate]: ASSY,MAIN,ELEVATOR.iam:1 ↔ ANGLE,MOUNT,ELEVATOR.ipt:1
- [Insert]: ASSY,MAIN,ELEVATOR.iam:1 ↔ SPACER,SPROCKET,IDLER,ELEVATOR.ipt:1
- [Insert]: ASSY,MAIN,ELEVATOR.iam:1 ↔ SPACER,SPROCKET,IDLER,ELEVATOR.ipt:1
- [Flush]: ASSY,MAIN,ELEVATOR.iam:1 ↔ 22.ipt:1
- [Insert]: ASSY,MAIN,ELEVATOR.iam:1 ↔ SPACER,SPROCKET,IDLER,ELEVATOR.ipt:2
- [Insert]: ASSY,MAIN,ELEVATOR.iam:1 ↔ SPACER,SPROCKET,IDLER,ELEVATOR.ipt:2
- Mate:223: BellyPanTop.ipt:1 ↔ PLATE,MOUNT,DRIVE,ELEVATOR.ipt:1
- Mate:224: ANGLE,MOUNT,ELEVATOR.ipt:1 ↔ PLATE,MOUNT,DRIVE,ELEVATOR.ipt:1
- Mate:226: PLATE,BEARING,DRIVE,ELEVATOR.ipt:1 ↔ PLATE,MOUNT,DRIVE,ELEVATOR.ipt:1
- Mate:227: 22.ipt:1 ↔ PLATE,BEARING,DRIVE,ELEVATOR.ipt:1
- Mate:228: PLATE,BEARING,DRIVE,ELEVATOR.ipt:1 ↔ PLATE,MOUNT,DRIVE,ELEVATOR.ipt:1
- Mate:229: PLATE,BEARING,DRIVE,ELEVATOR.ipt:1 ↔ PLATE,MOUNT,DRIVE,ELEVATOR.ipt:1
- Mate:230: PLATE,BEARING,DRIVE,ELEVATOR.ipt:2 ↔ PLATE,MOUNT,DRIVE,ELEVATOR.ipt:1
- Mate:231: PLATE,BEARING,DRIVE,ELEVATOR.ipt:2 ↔ PLATE,MOUNT,DRIVE,ELEVATOR.ipt:1
- Mate:232: PLATE,BEARING,DRIVE,ELEVATOR.ipt:2 ↔ PLATE,MOUNT,DRIVE,ELEVATOR.ipt:1
- Insert:49: PLATE,BEARING,DRIVE,ELEVATOR.ipt:2 ↔ PURCHASED,HEX_BEARING.ipt:1
- Insert:50: PLATE,BEARING,DRIVE,ELEVATOR.ipt:1 ↔ PURCHASED,HEX_BEARING.ipt:2
- Mate:233: 22.ipt:2 ↔ PLATE,BEARING,DRIVE,ELEVATOR.ipt:2
- Mate:234: PLATE,BEARING,DRIVE,ELEVATOR.ipt:2 ↔ SHAFT,HEX,0.500in,DRIVE,ELEVATOR.ipt:1
- Angle:4 (0 deg): 22.ipt:2 ↔ SHAFT,HEX,0.500in,DRIVE,ELEVATOR.ipt:1
- Angle:5 (0 deg): PURCHASED,HEX_BEARING.ipt:1 ↔ SHAFT,HEX,0.500in,DRIVE,ELEVATOR.ipt:1
- Angle:6 (0 deg): 22.ipt:1 ↔ SHAFT,HEX,0.500in,DRIVE,ELEVATOR.ipt:1
- Angle:7 (0 deg): PURCHASED,HEX_BEARING.ipt:2 ↔ SHAFT,HEX,0.500in,DRIVE,ELEVATOR.ipt:1
- [Flush]: ASSY,MAIN,ELEVATOR.iam:1 ↔ 22.ipt:2
- [Mate]: ASSY,MAIN,ELEVATOR.iam:1 ↔ PLATE,SIDE,BRACE,LEFT,ELEVATOR.ipt:1
- [Mate]: ASSY,MAIN,ELEVATOR.iam:1 ↔ PLATE,SIDE,BRACE,LEFT,ELEVATOR.ipt:1
- [Mate]: ASSY,MAIN,ELEVATOR.iam:1 ↔ 22.ipt:1
- Flush:14 (-15.875 mm): 22.ipt:2 ↔ SHAFT,HEX,0.500in,DRIVE,ELEVATOR.ipt:1
- Flush:17 (457.2 mm): MAXTube-2x1-Holes.ipt:2
- [Mate]: ASSY,MAIN,ELEVATOR.iam:1 ↔ PLATE,SIDE,BRACE,LEFT,ELEVATOR.ipt:1
- [Mate]: ASSY,MAIN,ELEVATOR.iam:1 ↔ PLATE,SIDE,BRACE,RIGHT,ELEVATOR.ipt:1
- [Mate]: ASSY,MAIN,ELEVATOR.iam:1 ↔ PLATE,SIDE,BRACE,RIGHT,ELEVATOR.ipt:1
- [Mate]: ASSY,MAIN,ELEVATOR.iam:1 ↔ PLATE,SIDE,BRACE,RIGHT,ELEVATOR.ipt:1
- Mate:271: MAXTube-2x1-Holes.ipt:4 ↔ PLATE,SIDE,BRACE,LEFT,ELEVATOR.ipt:1
- Mate:272: MAXTube-2x1-Holes.ipt:1 ↔ PLATE,SIDE,BRACE,RIGHT,ELEVATOR.ipt:1
- [Mate]: ASSY,MAIN,ELEVATOR.iam:1 ↔ TURNBUCKLE,0.25IN_CLEVIS.iam:1
- [Mate]: ASSY,MAIN,ELEVATOR.iam:1 ↔ TURNBUCKLE,0.25IN_CLEVIS.iam:1
- [Mate]: ASSY,MAIN,ELEVATOR.iam:1 ↔ TURNBUCKLE,0.25IN_CLEVIS.iam:2
- [Mate]: ASSY,MAIN,ELEVATOR.iam:1 ↔ TURNBUCKLE,0.25IN_CLEVIS.iam:2
- Mate:285: PLATE,BRACE,HORISONTAL,TOP,ELEVATOR.ipt:1 ↔ PLATE,TURNBUCKLE,TENSIONER,CHAIN.ipt:1
- Mate:286: PLATE,BRACE,HORISONTAL,TOP,ELEVATOR.ipt:1 ↔ PLATE,TURNBUCKLE,TENSIONER,CHAIN.ipt:2
- Mate:289: PLATE,BRACE,HORISONTAL,TOP,ELEVATOR.ipt:1 ↔ PLATE,SIDE,BRACE,LEFT,ELEVATOR.ipt:1
- Mate:290: PLATE,BRACE,HORISONTAL,TOP,ELEVATOR.ipt:1 ↔ PLATE,SIDE,BRACE,LEFT,ELEVATOR.ipt:1
- Mate:291: PLATE,BRACE,HORISONTAL,TOP,ELEVATOR.ipt:1 ↔ PLATE,SIDE,BRACE,LEFT,ELEVATOR.ipt:1
- [Mate]: ASSY,MAIN,ELEVATOR.iam:1 ↔ 22.ipt:2
- Mate:295: PLATE,BRACE,HORISONTAL,TOP,ELEVATOR.ipt:1 ↔ PLATE,TURNBUCKLE,TENSIONER,CHAIN.ipt:2
- Mate:296: PLATE,BRACE,HORISONTAL,TOP,ELEVATOR.ipt:1 ↔ PLATE,TURNBUCKLE,TENSIONER,CHAIN.ipt:1
- Flush:19: ASSY,MAIN,ELEVATOR.iam:1 ↔ STAGE1,ELEVATOR.iam:1
- Mate:297: ASSY,MAIN,ELEVATOR.iam:1 ↔ STAGE1,ELEVATOR.iam:1
- STAGE1 LOWER LIMIT [Mate]: STAGE1,ELEVATOR.iam:1 ↔ ANGLE,MOUNT,ELEVATOR.ipt:1
- STAGE1 UPPER LIMIT [Mate]: ASSY,MAIN,ELEVATOR.iam:1 ↔ STAGE1,ELEVATOR.iam:1
- STAGE1 MIN [Mate]: STAGE1,ELEVATOR.iam:1 ↔ ANGLE,MOUNT,ELEVATOR.ipt:1
- STAGE1 MAX [Mate] (3.175 mm): ASSY,MAIN,ELEVATOR.iam:1 ↔ STAGE1,ELEVATOR.iam:1
- Mate:308: BellyPanTop.ipt:1 ↔ ANGLE,MOUNT,ELEVATOR,MIRR.ipt:1
- Mate:309: MAXTube-2x1-Holes.ipt:2 ↔ ANGLE,MOUNT,ELEVATOR,MIRR.ipt:1
- Mate:310: MAXTube-2x1-Holes.ipt:2 ↔ ANGLE,MOUNT,ELEVATOR,MIRR.ipt:1
- Mate:311: ASSY,MAIN,ELEVATOR.iam:1 ↔ ANGLE,MOUNT,ELEVATOR,MIRR.ipt:1
- Mate:312: MAXTube-2x1-Holes.ipt:3 ↔ ANGLE,MOUNT,ELEVATOR,MIRR.ipt:1
- Mate:313: MAXTube-2x1-Holes.ipt:3 ↔ ANGLE,MOUNT,ELEVATOR,MIRR.ipt:1
- Mate:314: ASSY,MAIN,ELEVATOR.iam:1 ↔ ANGLE,MOUNT,ELEVATOR,MIRR.ipt:1
- Mate:315: ASSY,MAIN,ELEVATOR.iam:1 ↔ ANGLE,MOUNT,ELEVATOR,MIRR.ipt:1
- Mate:320: BellyPanTop.ipt:1 ↔ PLATE,MOUNT,BATTERY,BOT.ipt:1
- Flush:323 (146.05 mm): FABRIC,BUMPERS.ipt:1
- Mate:335 (3.175 mm): FABRIC,BUMPERS.ipt:1 ↔ PLATE,SIDE,BRACE,LEFT,ELEVATOR.ipt:1
- Mate:336 (6.35 mm): FABRIC,BUMPERS.ipt:1 ↔ MAXTube-2x1-Holes.ipt:3
- Mate:349: BellyPanTop.ipt:1 ↔ PLATE,MOUNT,BATTERY,TOP.ipt:1
- Mate:350: BellyPanTop.ipt:1 ↔ PLATE,MOUNT,BATTERY,TOP.ipt:1
- Mate:351: PLATE,MOUNT,BATTERY,BOT.ipt:1 ↔ PLATE,MOUNT,BATTERY,TOP.ipt:1
- Mate:352: PLATE,MOUNT,BATTERY,BOT.ipt:1 ↔ PLATE,MOUNT,BATTERY,TOP.ipt:1
- Mate:353: BellyPanBot.ipt:1 ↔ MAXTube-2x1-Holes.ipt:4
- Mate:354: BellyPanBot.ipt:1 ↔ MAXTube-2x1-Holes.ipt:4
- Mate:356 (19.05 mm): PLATE,MOUNT,BATTERY,TOP.ipt:1 ↔ BATTERY,12V.ipt:1
- Mate:357: MOUNT,STRAP,BATTERY.ipt:1 ↔ PLATE,MOUNT,BATTERY,TOP.ipt:1
- Mate:358: MOUNT,STRAP,BATTERY.ipt:1 ↔ PLATE,MOUNT,BATTERY,TOP.ipt:1
- Mate:359: MOUNT,STRAP,BATTERY.ipt:1 ↔ PLATE,MOUNT,BATTERY,TOP.ipt:1
- Mate:363: MOUNT,SPRING,ELEVATOR:1 ↔ ASSY,MAIN,ELEVATOR.iam:1
- Mate:362: MOUNT,SPRING,ELEVATOR:1 ↔ ASSY,MAIN,ELEVATOR.iam:1
- Mate:364: 9293K119_Constant-Force Spring:1 ↔ MOUNT,SPRING,ELEVATOR:1
- Mate:365 (1.5875 mm): 9293K119_Constant-Force Spring:1 ↔ MOUNT,SPRING,ELEVATOR:1
- Mate:366: MOUNT,SPRING,ELEVATOR:1 ↔ ASSY,MAIN,ELEVATOR.iam:1
- Mate:367: MOUNT,SPRING,ELEVATOR,MIRR:1 ↔ ASSY,MAIN,ELEVATOR.iam:1
- Mate:368: MOUNT,SPRING,ELEVATOR,MIRR:1 ↔ ASSY,MAIN,ELEVATOR.iam:1
- Mate:369: MOUNT,SPRING,ELEVATOR,MIRR:1 ↔ ASSY,MAIN,ELEVATOR.iam:1
- Mate:370: 9293K119_Constant-Force Spring:2 ↔ MOUNT,SPRING,ELEVATOR,MIRR:1
- Mate:371 (1.5875 mm): 9293K119_Constant-Force Spring:2 ↔ MOUNT,SPRING,ELEVATOR,MIRR:1
- Flush:329: ANGLE,MOUNT,ELEVATOR,MIRR.ipt:1 ↔ PLATE,MOUNT,DRIVE,ELEVATOR.ipt:1
- [Mate]: CONTROLS,MOTOR,NEO,550:3 ↔ VersaPlanetary v2 Dual Stage 10_1 with RS 550 (1):1
- [Mate]: CONTROLS,MOTOR,NEO,550:3 ↔ VersaPlanetary v2 Dual Stage 10_1 with RS 550 (1):1
- [Mate]: CONTROLS,MOTOR,NEO,550:4 ↔ VersaPlanetary v2 Dual Stage 10_1 with RS 550 (1):2
- [Mate]: CONTROLS,MOTOR,NEO,550:4 ↔ VersaPlanetary v2 Dual Stage 10_1 with RS 550 (1):2
- Mate:469: VersaPlanetary v2 Dual Stage 10_1 with RS 550 (1):2 ↔ PLATE,MOUNT,DRIVE,ELEVATOR.ipt:1
- Mate:470: VersaPlanetary v2 Dual Stage 10_1 with RS 550 (1):2 ↔ PLATE,MOUNT,DRIVE,ELEVATOR.ipt:1
- Mate:471: VersaPlanetary v2 Dual Stage 10_1 with RS 550 (1):2 ↔ PLATE,MOUNT,DRIVE,ELEVATOR.ipt:1
- Mate:472: VersaPlanetary v2 Dual Stage 10_1 with RS 550 (1):1 ↔ PLATE,MOUNT,DRIVE,ELEVATOR.ipt:1
- Mate:473: VersaPlanetary v2 Dual Stage 10_1 with RS 550 (1):1 ↔ PLATE,MOUNT,DRIVE,ELEVATOR.ipt:1
- Mate:474: VersaPlanetary v2 Dual Stage 10_1 with RS 550 (1):1 ↔ PLATE,MOUNT,DRIVE,ELEVATOR.ipt:1
- Angle:11 (15 deg): BellyPanTop.ipt:1 ↔ feeder_bottom_plate:1
- Mate:490: feeder_bottom_plate:1 ↔ hopper_back:1
- Mate:491: feeder_bottom_plate:1 ↔ hopper_back:1
- Mate:492: feeder_bottom_plate:1 ↔ hopper_back:1
- Mate:493: hopper_back:1 ↔ hopper_side_bracket:1
- Mate:494: hopper_back:1 ↔ hopper_side_bracket:1
- Mate:495: hopper_back:1 ↔ hopper_side_bracket:1
- Mate:496: hopper_side_l:1 ↔ hopper_side_bracket:1
- Mate:497: hopper_side_l:1 ↔ hopper_side_bracket:1
- Mate:498: hopper_side_l:1 ↔ hopper_side_bracket:1
- Mate:499: hopper_back:1 ↔ hopper_side_bracket:2
- Mate:500: hopper_back:1 ↔ hopper_side_bracket:2
- Mate:501: hopper_back:1 ↔ hopper_side_bracket:2
- Mate:502: hopper_side_r:1 ↔ hopper_side_bracket:2
- Mate:503: hopper_side_r:1 ↔ hopper_side_bracket:2
- Mate:504: hopper_side_r:1 ↔ hopper_side_bracket:2
- Flush:330 (464.82 mm)
- Flush:331 (-57.15 mm)
- Mate:507: feeder_bottom_plate:1 ↔ feeder_guide_plate:1
- Mate:512: feeder_bottom_plate:1 ↔ feeder_guide_plate_MIR:1
- Mate:519 (57.15 mm): feeder_bottom_plate:1 ↔ Coral:1
- Mate:520 (58.7375 mm): feeder_guide_plate_MIR:1 ↔ Coral:1
- [Mate]: CONTROLS,MOTOR,NEO,550:5 ↔ VersaPlanetary v2 Dual Stage 10_1 with RS 550 (1):3
- [Mate]: CONTROLS,MOTOR,NEO,550:5 ↔ VersaPlanetary v2 Dual Stage 10_1 with RS 550 (1):3
- Mate:534: feeder_bottom_plate:1 ↔ VersaPlanetary v2 Dual Stage 10_1 with RS 550 (1):3
- Angle:12 (180 deg): ANGLE,MOUNT,ELEVATOR,MIRR.ipt:1 ↔ feeder_bottom_plate:1
- Flush:333: feeder_bottom_plate:1 ↔ coral_guide:1
- Mate:537: feeder_bottom_plate:1 ↔ coral_guide:1
- Flush:334: feeder_bottom_plate:1 ↔ coral_guide_MIR:1
- Mate:539: feeder_bottom_plate:1 ↔ coral_guide_MIR:1
- Mate:540 (69.85 mm): coral_guide:1 ↔ coral_guide_MIR:1
- Flush:335 (11.1125 mm): feeder_bottom_plate:1 ↔ coral_guide:1
- Mate:541: BellyPanTop.ipt:1 ↔ feeder_front_support:1
- Mate:542: BellyPanTop.ipt:1 ↔ MAXTube-2x1-Holes.ipt:2
- Mate:543: MAXTube-2x1-Holes.ipt:2 ↔ feeder_front_support:1
- Mate:544: BellyPanTop.ipt:1 ↔ feeder_front_support:1
- Mate:545: feeder_bottom_plate:1 ↔ hopper_back_support:1
- Mate:546: feeder_bottom_plate:1 ↔ hopper_back_support:1
- Mate:547: feeder_bottom_plate:1 ↔ hopper_back_support:1
- Mate:548: BellyPanTop.ipt:1 ↔ hopper_back_support:1
- Flush:336: BellyPanTop.ipt:1 ↔ hopper_back_support:1
- Mate:549: BellyPanTop.ipt:1 ↔ hopper_back_support:1
- Flush:337: ANGLE,MOUNT,ELEVATOR.ipt:1 ↔ feeder_side_support_r:1
- Mate:550: ANGLE,MOUNT,ELEVATOR,MIRR.ipt:1 ↔ feeder_side_support_l:1
- Mate:551: ANGLE,MOUNT,ELEVATOR,MIRR.ipt:1 ↔ feeder_side_support_l:1
- Mate:552: ANGLE,MOUNT,ELEVATOR,MIRR.ipt:1 ↔ feeder_side_support_l:1
- Mate:553: feeder_side_support_r:1 ↔ feeder_middle_brace:1
- Mate:554: feeder_side_support_r:1 ↔ feeder_middle_brace:1
- Mate:555: feeder_side_support_r:1 ↔ feeder_middle_brace:1
- Mate:556: ANGLE,MOUNT,ELEVATOR.ipt:1 ↔ feeder_side_support_r:1
- Mate:557: 2_1-2_hex_shaft:1 ↔ PURCHASED,HEX_BEARING:3
- Mate:558: 2_1-2_hex_shaft:1 ↔ PURCHASED,HEX_BEARING:3
- Flush:340: 2_1-2_hex_shaft:1 ↔ PURCHASED,HEX_BEARING:3
- [Mate]: 2_1-2_hex_shaft:2 ↔ PURCHASED,HEX_BEARING:4
- [Mate]: 2_1-2_hex_shaft:2 ↔ PURCHASED,HEX_BEARING:4
- [Flush]: 2_1-2_hex_shaft:2 ↔ PURCHASED,HEX_BEARING:4
- Mate:561: 2_1-2_hex_shaft:1 ↔ am-5123 5IN 500IN Hex Bore Compliant Star:3
- Mate:562: 2_1-2_hex_shaft:1 ↔ am-5123 5IN 500IN Hex Bore Compliant Star:3
- Mate:573: PURCHASED,HEX_BEARING:3 ↔ am-5123 5IN 500IN Hex Bore Compliant Star:3
- Mate:577: feeder_bottom_plate:1 ↔ feeder_guide_plate:1
- Mate:578: feeder_bottom_plate:1 ↔ feeder_guide_plate_MIR:1
- [Mate]: 2_1-2_hex_shaft:3 ↔ PURCHASED,HEX_BEARING:5
- [Mate]: 2_1-2_hex_shaft:3 ↔ PURCHASED,HEX_BEARING:5
- [Flush]: 2_1-2_hex_shaft:3 ↔ PURCHASED,HEX_BEARING:5
- [Mate]: 2_1-2_hex_shaft:3 ↔ am-5123 5IN 500IN Hex Bore Compliant Star:5
- [Mate]: 2_1-2_hex_shaft:3 ↔ am-5123 5IN 500IN Hex Bore Compliant Star:5
- [Mate]: PURCHASED,HEX_BEARING:5 ↔ am-5123 5IN 500IN Hex Bore Compliant Star:5
- [Mate]: 2_1-2_hex_shaft:4 ↔ PURCHASED,HEX_BEARING:6
- [Mate]: 2_1-2_hex_shaft:4 ↔ PURCHASED,HEX_BEARING:6
- [Flush]: 2_1-2_hex_shaft:4 ↔ PURCHASED,HEX_BEARING:6
- [Mate]: CONTROLS,MOTOR,NEO,550:6 ↔ VersaPlanetary v2 Dual Stage 10_1 with RS 550 (1):4
- [Mate]: CONTROLS,MOTOR,NEO,550:6 ↔ VersaPlanetary v2 Dual Stage 10_1 with RS 550 (1):4
- Mate:605: feeder_bottom_plate:1 ↔ VersaPlanetary v2 Dual Stage 10_1 with RS 550 (1):4
- Mate:608: feeder_bottom_plate:1 ↔ Bolt_Spacer:1
- Mate:609: feeder_bottom_plate:1 ↔ Bolt_Spacer:1
- Mate:610: feeder_bottom_plate:1 ↔ Bolt_Spacer:2
- Mate:611: feeder_bottom_plate:1 ↔ Bolt_Spacer:2
- [Mate]: CONTROLS,SPARK_MAX:9 ↔ COVER,SPARKMAX:9
- [Mate]: CONTROLS,SPARK_MAX:9 ↔ COVER,SPARKMAX:9
- [Mate]: CONTROLS,SPARK_MAX:9 ↔ COVER,SPARKMAX:9
- [Mate]: CONTROLS,SPARK_MAX:10 ↔ COVER,SPARKMAX:10
- [Mate]: CONTROLS,SPARK_MAX:10 ↔ COVER,SPARKMAX:10
- [Mate]: CONTROLS,SPARK_MAX:10 ↔ COVER,SPARKMAX:10
- Mate:624: feeder_side_support_r:1 ↔ COVER,SPARKMAX:9
- Mate:625: feeder_side_support_r:1 ↔ COVER,SPARKMAX:9
- Mate:626: feeder_side_support_r:1 ↔ CONTROLS,SPARK_MAX:9
- Mate:627: feeder_side_support_l:1 ↔ COVER,SPARKMAX:10
- Mate:628: feeder_side_support_l:1 ↔ COVER,SPARKMAX:10
- Mate:629: feeder_side_support_l:1 ↔ CONTROLS,SPARK_MAX:10
- Mate:630 (57.15 mm): feeder_bottom_plate:1 ↔ Coral:1
- Mate:631: feeder_bottom_plate:1 ↔ VersaPlanetary v2 Dual Stage 10_1 with RS 550 (1):3
- Mate:632: feeder_bottom_plate:1 ↔ VersaPlanetary v2 Dual Stage 10_1 with RS 550 (1):3
- Mate:633: feeder_bottom_plate:1 ↔ VersaPlanetary v2 Dual Stage 10_1 with RS 550 (1):4
- Mate:634: feeder_bottom_plate:1 ↔ VersaPlanetary v2 Dual Stage 10_1 with RS 550 (1):4
- Mate:636: PURCHASED,HEX_BEARING:11 ↔ 2_1-2_hex_shaft:6
- Mate:637: PURCHASED,HEX_BEARING:11 ↔ 2_1-2_hex_shaft:6
- Flush:349: PURCHASED,HEX_BEARING:11 ↔ 2_1-2_hex_shaft:6
- Flush:350: 2_1-2_hex_shaft:6 ↔ PURCHASED,HEX_BEARING:14
- Mate:638: 2_1-2_hex_shaft:6 ↔ PURCHASED,HEX_BEARING:14
- Mate:639: 2_1-2_hex_shaft:6 ↔ PURCHASED,HEX_BEARING:14
- Flush:351: 2_1-2_hex_shaft:5 ↔ PURCHASED,HEX_BEARING:12
- Mate:640: 2_1-2_hex_shaft:5 ↔ PURCHASED,HEX_BEARING:12
- Mate:641: 2_1-2_hex_shaft:5 ↔ PURCHASED,HEX_BEARING:12
- Flush:352: 2_1-2_hex_shaft:5 ↔ PURCHASED,HEX_BEARING:13
- Mate:642: 2_1-2_hex_shaft:5 ↔ PURCHASED,HEX_BEARING:13
- Mate:643: 2_1-2_hex_shaft:5 ↔ PURCHASED,HEX_BEARING:13
- Mate:644: feeder_guide_plate:1 ↔ PURCHASED,HEX_BEARING:12
- Mate:645: feeder_guide_plate:1 ↔ PURCHASED,HEX_BEARING:12
- Mate:646: feeder_bottom_plate:1 ↔ PURCHASED,HEX_BEARING:8
- Mate:647: feeder_bottom_plate:1 ↔ PURCHASED,HEX_BEARING:8
- Mate:648: feeder_bottom_plate:1 ↔ PURCHASED,HEX_BEARING:7
- Mate:649: feeder_bottom_plate:1 ↔ PURCHASED,HEX_BEARING:7
- Mate:650: feeder_guide_plate:1 ↔ PURCHASED,HEX_BEARING:4
- Mate:651: feeder_guide_plate:1 ↔ PURCHASED,HEX_BEARING:4